# Autodesk Inventor assembly: Cartridge Enclosure1460102
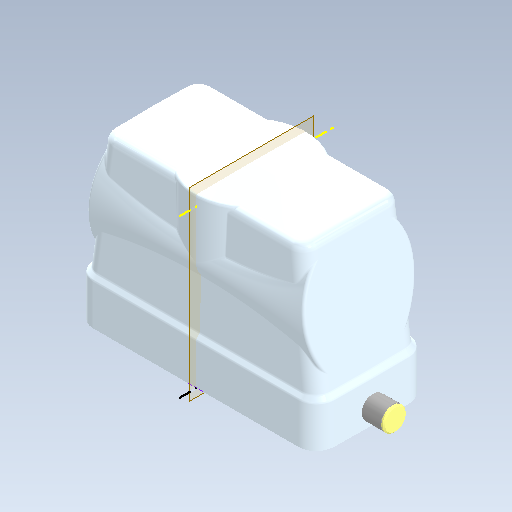
[picture p0: Inventor's stored thumbnail of the model, 512x512]
Saved by Autodesk Inventor 2021 (Build 250183000, 183)
## iProperties
Created: 2012-08-01
Part Number: Cartridge Enclosure1460102
Description: SolidDesigner STEP Export
Document SubType Name: Assembly
Designer: jgray
Title: 1460102.stp
## Documents named in this file (2)
- M:\Printed Electronics\Gas Sensors\Prototypes\Prototype II - Cartridge Reader\Full Cart Interface V3 28-5-20\Workspaces\Workspace\Workspaces\Workspace\Externally supplied Parts\Cart Enclosure\Cartridge Enclosure1460102.iam
- M:\Printed Electronics\Gas Sensors\Prototypes\Prototype II - Cartridge Reader\Full Cart Interface V3 28-5-20\Workspaces\Workspace\Workspaces\Workspace\Externally supplied Parts\Cart Enclosure\Cartridge Enclosure1460102.ipt
## Components (1 placed, 1 different names)
1. 1 — Mate:1, Mate:2, Mate:3
## Relationships (3: Mate 3)
- Mate:1: 1
- Mate:2: 1
- Mate:3: 1
